# Autodesk Inventor assembly: писюны
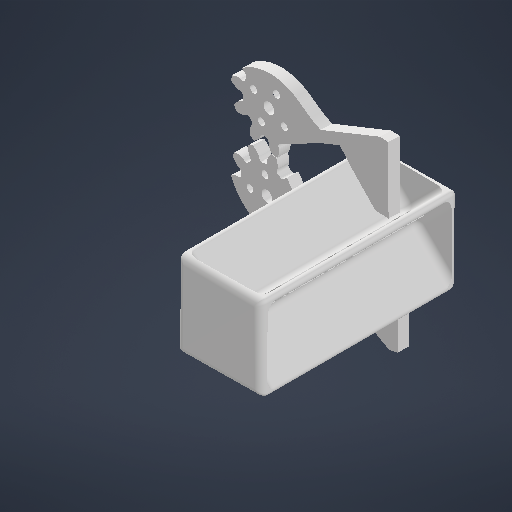
[picture p0: Inventor's stored thumbnail of the model, 512x512]
Saved by Autodesk Inventor 2025 (Build 290162000, 162)
## iProperties
Created: 2024-12-28
Part Number: писюны
Document SubType Name: Assembly
Designer: Phantom
Author: Phantom
## Documents named in this file (4)
- C:\Users\Phantom\Desktop\Phantom16950\писюны.iam
- C:\Users\Phantom\Downloads\am-5401 Sample\am-5401 Sample.ipt
- C:\Users\Phantom\Desktop\Phantom16950\писюн.ipt
- C:\Users\Phantom\Desktop\Phantom16950\писюн 2_MIR.ipt
## Components (3 placed, 3 different names)
1. am-5401 Sample:1
2. писюн:1 — Заподлицо:1
3. писюн 2_MIR:1 — Заподлицо:1
## Relationships (1: Flush 1)
- Заподлицо:1 [Flush]: писюн:1 ↔ писюн 2_MIR:1
